# Autodesk Inventor assembly: racked
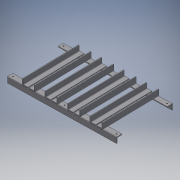
[picture p0: Inventor's stored thumbnail of the model, 180x180]
Saved by Autodesk Inventor 2017 (Build 210142000, 142)
## iProperties
Created: 2018-10-17
Part Number: racked
Document SubType Name: Assembly
Designer: ddeboer
Author: ddeboer
## Documents named in this file (3)
- C:\Users\ddeboer\Desktop\snap_holder\ladder.iam
- C:\Users\ddeboer\Desktop\snap_holder\channel.ipt
- C:\Users\ddeboer\Desktop\snap_holder\uchannel.ipt
## Components (10 placed, 2 different names)
1. channel:1 — Flush:5, Flush:6, Flush:7, Flush:8
2. channel:2 — Mate:3, Mate:4, Flush:6, Flush:7, Flush:9
3. uchannel:1 — Flush:5, Mate:4, Mate:5, Flush:9
4. uchannel:2 — Mate:3, Flush:8, Mate:5
5. uchannel:3
6. uchannel:4
7. uchannel:5
8. uchannel:6
9. uchannel:7
10. uchannel:8
## Component patterns: (4 elements, first: uchannel:1 + uchannel:2)
## Relationships (8: Flush 5, Mate 3)
- Flush:5: channel:1 ↔ uchannel:1
- Mate:3: channel:2 ↔ uchannel:2
- Mate:4: channel:2 ↔ uchannel:1
- Flush:6: channel:1 ↔ channel:2
- Flush:7: channel:1 ↔ channel:2
- Flush:8: channel:1 ↔ uchannel:2
- Mate:5 (50.8 mm): uchannel:1 ↔ uchannel:2
- Flush:9: channel:2 ↔ uchannel:1
